# Autodesk Inventor assembly: Assembly roller
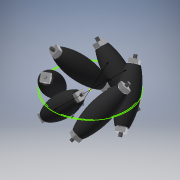
[picture p0: Inventor's stored thumbnail of the model, 180x180]
Saved by Autodesk Inventor 2018 (Build 220112000, 112)
## iProperties
Created: 2017-08-22
Part Number: Assembly roller
Document SubType Name: Assembly
Designer: P445885
Mass: 3322.13 g
Surface Area: 5085.83 cm^2
Volume: 1748.22 cm^3
Density: 1.9003 g/cm^3
Author: P445885
## Documents named in this file (12)
- E:\advanced diploma\Project\Autonomous\Assembly roller.iam
- E:\advanced diploma\Project\Autonomous\roller 8-19-6 bearing.ipt
- C:\Users\P445885\Documents\Inventor\Content Center Files\R2018\en-US\DIN 625 SKF(4)\DIN 625 SKF - SKF 619_8-2Z.ipt
- E:\advanced diploma\Project\Autonomous\rubber.ipt
- E:\advanced diploma\Project\Autonomous\axial.ipt
- E:\advanced diploma\Project\Autonomous\washer.ipt
- E:\advanced diploma\Project\Autonomous\Assembly roller\AIP\FEA\c8vujv74w.fins
- E:\advanced diploma\Project\Autonomous\Assembly roller\AIP\FEA\c8vujv74w.fsat
- E:\advanced diploma\Project\Autonomous\Assembly roller\AIP\FEA\c8vujv74w.ftes
- E:\advanced diploma\Project\Autonomous\Assembly roller\AIP\FEA\c8vujv74w.fwiz
- E:\advanced diploma\Project\Autonomous\Assembly roller\AIP\FEA\c8vujv79c.fmsh
- E:\advanced diploma\Project\Autonomous\Assembly roller\AIP\FEA\c8vujv79d.fres
## Components (42 placed, 5 different names)
1. roller 8-19-6 bearing:1 — Mate:1, Mate:2, Angle:1
2. rubber:1 — Insert:1
3. DIN 625 SKF- with two Z shields SKF 619/8-2Z:1 — Mate:3, Mate:4
4. DIN 625 SKF- with two Z shields SKF 619/8-2Z:2 — Mate:5, Mate:6
5. axial:1 — Mate:7, Mate:8, Mate:9, Mate:11
6. washer:1 — Mate:9, Mate:10
7. washer:2 — Mate:11, Mate:12
8. roller 8-19-6 bearing:2 — Mate:3, Mate:4, Mate:5, Mate:6
9. rubber:2 — Mate:12
10. DIN 625 SKF- with two Z shields SKF 619/8-2Z:3
11. DIN 625 SKF- with two Z shields SKF 619/8-2Z:8
12. axial:2
13. washer:3
14. washer:8
15. roller 8-19-6 bearing:3 — Insert:1
16. rubber:3
17. DIN 625 SKF- with two Z shields SKF 619/8-2Z:4
18. DIN 625 SKF- with two Z shields SKF 619/8-2Z:9 — Mate:8
19. axial:3
20. washer:4
21. washer:9
22. roller 8-19-6 bearing:4 — Mate:7, Mate:10
23. rubber:4
24. DIN 625 SKF- with two Z shields SKF 619/8-2Z:5
25. DIN 625 SKF- with two Z shields SKF 619/8-2Z:10
26. axial:4
27. washer:5
28. washer:10
29. roller 8-19-6 bearing:5
30. rubber:5
31. DIN 625 SKF- with two Z shields SKF 619/8-2Z:6
32. DIN 625 SKF- with two Z shields SKF 619/8-2Z:11
33. axial:5
34. washer:6
35. washer:11
36. roller 8-19-6 bearing:6
37. rubber:6
38. DIN 625 SKF- with two Z shields SKF 619/8-2Z:7
39. DIN 625 SKF- with two Z shields SKF 619/8-2Z:12
40. axial:6
41. washer:7
42. washer:12
## Component patterns: (6 elements, first: roller 8-19-6 bearing:1 + rubber:1 + DIN 625 SKF- with two Z shields SKF 619/8-2Z:1 + DIN 625 SKF- with two Z shields SKF 619/8-2Z:2 + axial:1 + washer:1 + washer:2)
## Relationships (14: Mate 12, Angle 1, Insert 1)
- Mate:1: roller 8-19-6 bearing:1
- Mate:2 (75 mm): roller 8-19-6 bearing:1
- Angle:1 (45 deg): roller 8-19-6 bearing:1
- Mate:3: DIN 625 SKF- with two Z shields SKF 619/8-2Z:1 ↔ roller 8-19-6 bearing:2
- Mate:4: DIN 625 SKF- with two Z shields SKF 619/8-2Z:1 ↔ roller 8-19-6 bearing:2
- Mate:5: DIN 625 SKF- with two Z shields SKF 619/8-2Z:2 ↔ roller 8-19-6 bearing:2
- Mate:6: DIN 625 SKF- with two Z shields SKF 619/8-2Z:2 ↔ roller 8-19-6 bearing:2
- Insert:1: rubber:1 ↔ roller 8-19-6 bearing:3
- Mate:7: axial:1 ↔ roller 8-19-6 bearing:4
- Mate:8 (-20 mm): axial:1 ↔ DIN 625 SKF- with two Z shields SKF 619/8-2Z:9
- Mate:9: axial:1 ↔ washer:1
- Mate:10 (1 mm): washer:1 ↔ roller 8-19-6 bearing:4
- Mate:11: axial:1 ↔ washer:2
- Mate:12 (1 mm): washer:2 ↔ rubber:2
## Named parameters: sa_0 = -73265.7, sa_1 = -42300, sa_2 = 6.11e-11
note: some values were not read from the file. Shown as the stored number, unit unknown: "sa_0", "sa_1", "sa_2".
